# Autodesk Inventor assembly: CompressionGrip
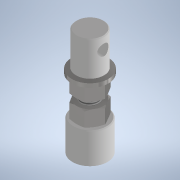
[picture p0: Inventor's stored thumbnail of the model, 180x180]
Saved by Autodesk Inventor 2020 (Build 240168000, 168)
## iProperties
Created: 2020-03-19
Part Number: CompressionGrip
Document SubType Name: Assembly
Designer: Naude Conradie
Author: Naude Conradie
## Documents named in this file (5)
- C:\Users\Naude Conradie\Desktop\Repository\Masters-Project\Models\Inventor\CompressionGripAssembly.iam
- C:\Users\Naude Conradie\Desktop\Repository\Masters-Project\Models\Inventor\CompressionGrip.ipt
- C:\Users\Naude Conradie\Desktop\Repository\Masters-Project\Models\Inventor\CompressionGripAttachment.ipt
- C:\Users\Naude Conradie\Documents\Inventor\Content Center Files\R2020\en-US\ANSI B 18.2.4.1 M(1)\ANSI B 18.2.4.1 M - M20 x 2,5Style 1.ipt
- C:\Users\Naude Conradie\Documents\Inventor\Content Center Files\R2020\en-US\IFI 542(1)\IFI 542 - 20(1).ipt
## Components (5 placed, 4 different names)
1. CompressionGrip:1 — Mate:1, Mate:2, Flush:1, Mate:4
2. CompressionGripAttachment:1 — Mate:1, Mate:2, Flush:1, Flush:2, Mate:3, Flush:3, Mate:5, Mate:6, Flush:4, Mate:7
3. Hex Nut Metric M20 x 2,5:1 — Flush:2, Mate:3, Mate:4
4. Hex Nut Metric M20 x 2,5:2 — Flush:4, Mate:7, Mate:8
5. Circular Washer (Metric) (IFI) 20:1 — Flush:3, Mate:5, Mate:6, Mate:8
## Relationships (12: Mate 8, Flush 4)
- Mate:1: CompressionGrip:1 ↔ CompressionGripAttachment:1
- Mate:2: CompressionGrip:1 ↔ CompressionGripAttachment:1
- Flush:1: CompressionGrip:1 ↔ CompressionGripAttachment:1
- Flush:2: CompressionGripAttachment:1 ↔ Hex Nut Metric M20 x 2,5:1
- Mate:3: CompressionGripAttachment:1 ↔ Hex Nut Metric M20 x 2,5:1
- Mate:4: CompressionGrip:1 ↔ Hex Nut Metric M20 x 2,5:1
- Flush:3: CompressionGripAttachment:1 ↔ Circular Washer (Metric) (IFI) 20:1
- Mate:5: CompressionGripAttachment:1 ↔ Circular Washer (Metric) (IFI) 20:1
- Mate:6: CompressionGripAttachment:1 ↔ Circular Washer (Metric) (IFI) 20:1
- Flush:4: CompressionGripAttachment:1 ↔ Hex Nut Metric M20 x 2,5:2
- Mate:7: CompressionGripAttachment:1 ↔ Hex Nut Metric M20 x 2,5:2
- Mate:8: Hex Nut Metric M20 x 2,5:2 ↔ Circular Washer (Metric) (IFI) 20:1
